# Autodesk Inventor assembly: leg5
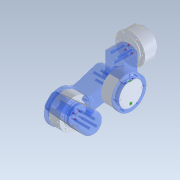
[picture p0: Inventor's stored thumbnail of the model, 180x180]
Saved by Autodesk Inventor 2020 (Build 240168000, 168)
## iProperties
Created: 2020-12-24
Part Number: leg5
Document SubType Name: Assembly
Designer: DELL
Author: DELL
## Documents named in this file (6)
- F:\SoftRobot2.0\Flexipod2.0\leg5_2020_12_24_11_46\leg5.2.iam
- F:\SoftRobot2.0\Flexipod2.0\RMD_X6_stator.ipt
- F:\SoftRobot2.0\Flexipod2.0\RMD_X6_rotor.ipt
- F:\SoftRobot2.0\Flexipod2.0\leg5_2020_12_24_11_46\shank_link.ipt
- F:\SoftRobot2.0\Flexipod2.0\leg5_2020_12_24_11_46\thigh_link_2.ipt
- F:\SoftRobot2.0\Flexipod2.0\leg5_2020_12_24_11_46\hip_link_2.ipt
## Components (9 placed, 5 different names)
1. RMD_X6_stator:1 — Mate:1, Flush:1, Mate:30, Mate:31, Flush:4
2. RMD_X6_rotor:1 — Mate:1, Flush:1, Mate:27, Mate:28, Mate:29
3. RMD_X6_stator:2 — Mate:2, Flush:2, Mate:16, Mate:18, Angle:1, Mate:24, Mate:25, Mate:26
4. RMD_X6_rotor:2 — Mate:2, Flush:2, Mate:17, Mate:19
5. RMD_X6_stator:3 — Mate:4, Mate:20, Mate:22, Mate:23
6. RMD_X6_rotor:3 — Mate:5, Mate:6
7. shank_link:1 — Mate:4, Mate:5, Mate:6
8. thigh_link_2:1 — Mate:16, Mate:17, Mate:18, Mate:19, Mate:20, Mate:22, Mate:23
9. hip_link_2:1 — Mate:24, Mate:25, Mate:26, Mate:27, Mate:28, Mate:29
## Relationships (26: Mate 21, Flush 4, Angle 1)
- Mate:1: RMD_X6_stator:1 ↔ RMD_X6_rotor:1
- Flush:1 (-3 mm): RMD_X6_stator:1 ↔ RMD_X6_rotor:1
- Mate:2: RMD_X6_stator:2 ↔ RMD_X6_rotor:2
- Flush:2 (-3 mm): RMD_X6_stator:2 ↔ RMD_X6_rotor:2
- [Mate]: RMD_X6_stator:3 ↔ RMD_X6_rotor:3
- [Flush] (-3 mm): RMD_X6_stator:3 ↔ RMD_X6_rotor:3
- Mate:4: RMD_X6_stator:3 ↔ shank_link:1
- Mate:5: RMD_X6_rotor:3 ↔ shank_link:1
- Mate:6: RMD_X6_rotor:3 ↔ shank_link:1
- Mate:16: RMD_X6_stator:2 ↔ thigh_link_2:1
- Mate:17: RMD_X6_rotor:2 ↔ thigh_link_2:1
- Mate:18: RMD_X6_stator:2 ↔ thigh_link_2:1
- Mate:19: RMD_X6_rotor:2 ↔ thigh_link_2:1
- Mate:20: RMD_X6_stator:3 ↔ thigh_link_2:1
- Mate:22: RMD_X6_stator:3 ↔ thigh_link_2:1
- Angle:1 (0 deg): RMD_X6_stator:2
- Mate:23: RMD_X6_stator:3 ↔ thigh_link_2:1
- Mate:24: RMD_X6_stator:2 ↔ hip_link_2:1
- Mate:25: RMD_X6_stator:2 ↔ hip_link_2:1
- Mate:26: RMD_X6_stator:2 ↔ hip_link_2:1
- Mate:27: RMD_X6_rotor:1 ↔ hip_link_2:1
- Mate:28: RMD_X6_rotor:1 ↔ hip_link_2:1
- Mate:29: RMD_X6_rotor:1 ↔ hip_link_2:1
- Mate:30: RMD_X6_stator:1
- Mate:31: RMD_X6_stator:1
- Flush:4: RMD_X6_stator:1
## Named parameters: d4_d2 = 0 mm, d5_d3 = -3 mm
